# Autodesk Inventor assembly: HbMRLFinger
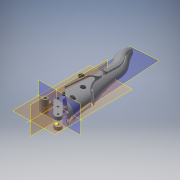
[picture p0: Inventor's stored thumbnail of the model, 180x180]
Saved by Autodesk Inventor 2017 (Build 210142000, 142)
## iProperties
Part Number: HbMRLFinger
Material: 一般
Document SubType Name: Assembly
Designer: sktom
Author: sktom
## Documents named in this file (7)
- D:\OneDrive\CAD\MAJ\hackberry\HACKberry-hardware\3D_69%\Inventor\HbHandForChild\HbFinger01ForChild\HbFinger01ForChild.iam
- D:\OneDrive\CAD\MAJ\hackberry\HACKberry-hardware\3D_69%\Inventor\HbHandForChild\HbFinger01ForChild\HbCouplerLinkCover03ForChild.ipt
- D:\OneDrive\CAD\MAJ\hackberry\HACKberry-hardware\3D_69%\Inventor\HbHandForChild\HbFinger01ForChild\HbCouplerLink02ForChild.ipt
- D:\OneDrive\CAD\MAJ\hackberry\HACKberry-hardware\3D_69%\Inventor\HbHandForChild\HbFinger01ForChild\HbMiddle-DistalPhalanx02ForChild.ipt
- D:\OneDrive\CAD\MAJ\hackberry\HACKberry-hardware\3D_69%\Inventor\HbHandForChild\HbFinger01ForChild\HbProximalPhalanx02ForChild.ipt
- D:\OneDrive\CAD\MAJ\hackberry\HACKberry-hardware\3D_69%\Inventor\HbHandForChild\HbFinger01ForChild\HbProximalPhalanxCover02ForChild.ipt
- D:\OneDrive\CAD\MAJ\hackberry\HACKberry-hardware\3D_69%\Inventor\HbHandForChild\HbFinger01ForChild\M2_L8.ipt
## Components (9 placed, 6 different names)
1. HbCouplerLinkCover03ForChild:1 — 挿入:1, 挿入:2
2. HbCouplerLink02ForChild:1 — 挿入:1, 挿入:2, 挿入:3, 挿入:8, 挿入:9
3. HbMiddle-DistalPhalanx02ForChild:1 — 挿入:3, 挿入:4
4. HbProximalPhalanx02ForChild:1 — 挿入:5, 挿入:6
5. HbProximalPhalanxCover02ForChild:1 — 挿入:4, 挿入:5, 挿入:6, 挿入:7, 挿入:10
6. M2_L8:1 — 挿入:7
7. M2_L8:2 — 挿入:9
8. M2_L8:3 — 挿入:8
9. M2_L8:4 — 挿入:10
## Relationships (10: Insert 10)
- 挿入:1 [Insert]: HbCouplerLinkCover03ForChild:1 ↔ HbCouplerLink02ForChild:1
- 挿入:2 [Insert]: HbCouplerLinkCover03ForChild:1 ↔ HbCouplerLink02ForChild:1
- 挿入:3 [Insert] (0.4 mm): HbCouplerLink02ForChild:1 ↔ HbMiddle-DistalPhalanx02ForChild:1
- 挿入:4 [Insert] (0.4 mm): HbMiddle-DistalPhalanx02ForChild:1 ↔ HbProximalPhalanxCover02ForChild:1
- 挿入:5 [Insert]: HbProximalPhalanx02ForChild:1 ↔ HbProximalPhalanxCover02ForChild:1
- 挿入:6 [Insert]: HbProximalPhalanx02ForChild:1 ↔ HbProximalPhalanxCover02ForChild:1
- 挿入:7 [Insert]: HbProximalPhalanxCover02ForChild:1 ↔ M2_L8:1
- 挿入:8 [Insert]: HbCouplerLink02ForChild:1 ↔ M2_L8:3
- 挿入:9 [Insert]: HbCouplerLink02ForChild:1 ↔ M2_L8:2
- 挿入:10 [Insert]: HbProximalPhalanxCover02ForChild:1 ↔ M2_L8:4
